# Autodesk Inventor assembly: Horizontal track
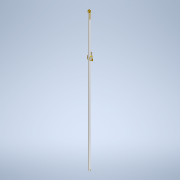
[picture p0: Inventor's stored thumbnail of the model, 180x180]
Saved by Autodesk Inventor 2022 (Build 260153000, 153)
## iProperties
RuleStatus: InUse
Created: 2021-12-23
Part Number: Horizontal track
Document SubType Name: Assembly
Designer: matte
Author: matte
## Documents named in this file (8)
- C:\Users\matte\Documents\GitHub\MDM-Homework\CAD\Horizontal track.iam
- C:\Users\matte\Documents\GitHub\MDM-Homework\CAD\Parts\Ground track\10-081.ipt
- C:\Users\matte\Documents\GitHub\MDM-Homework\CAD\Parts\Ground track\10-240.ipt
- C:\Users\matte\Documents\GitHub\MDM-Homework\CAD\Parts\Ground track\13-106.ipt
- C:\Users\matte\Documents\GitHub\MDM-Homework\CAD\Parts\Ground track\13-505.ipt
- C:\Users\matte\Documents\GitHub\MDM-Homework\CAD\Parts\Ground track\30-404.ipt
- C:\Users\matte\Documents\GitHub\MDM-Homework\CAD\Parts\Ground track\30-407.ipt
- C:\Users\matte\Documents\GitHub\MDM-Homework\CAD\Inventor Component Part Files\08-Linear Application\06-Linear Roller System\04-Components for Bearing Units\02-Bolts\30-006.ipt
## Components (10 placed, 7 different names)
1. 10-081:1 — Allineato:8, Coincidente:7, Allineato:9, Coincidente:8, Allineato:10, Allineato:12
2. 10-240:1 — Allineato:1, Allineato:3, Coincidente:1, Coincidente:2, Coincidente:3, Allineato:4, Allineato:5, Allineato:6, Allineato:12, Allineato:13
3. 13-106:1 — Allineato:1, Allineato:3, Coincidente:1, Coincidente:4, Coincidente:5
4. 13-505:1 — Allineato:5, Coincidente:4, Coincidente:5
5. 30-404:1 — Allineato:8, Coincidente:7, Allineato:9, Allineato:11, Allineato:13
6. 30-407:1 — Coincidente:9, Allineato:14, Allineato:15
7. 13-106:2 — Coincidente:2, Coincidente:3, Allineato:4, Coincidente:6, Allineato:7
8. 13-505:2 — Coincidente:6, Allineato:6, Allineato:7
9. 30-404:2 — Coincidente:8, Allineato:10, Allineato:11, Coincidente:9, Allineato:14, Allineato:15, Inserimento:1
10. 30-006:1 — Inserimento:1
## Relationships (24: Flush 14, Mate 9, Insert 1)
- Allineato:1 [Flush]: 10-240:1 ↔ 13-106:1
- Allineato:3 [Flush]: 10-240:1 ↔ 13-106:1
- Coincidente:1 [Mate]: 10-240:1 ↔ 13-106:1
- Coincidente:2 [Mate]: 10-240:1 ↔ 13-106:2
- Coincidente:3 [Mate]: 10-240:1 ↔ 13-106:2
- Allineato:4 [Flush]: 10-240:1 ↔ 13-106:2
- Allineato:5 [Flush]: 10-240:1 ↔ 13-505:1
- Coincidente:4 [Mate]: 13-106:1 ↔ 13-505:1
- Coincidente:5 [Mate]: 13-106:1 ↔ 13-505:1
- Coincidente:6 [Mate]: 13-106:2 ↔ 13-505:2
- Allineato:6 [Flush]: 10-240:1 ↔ 13-505:2
- Allineato:7 [Flush]: 13-106:2 ↔ 13-505:2
- Allineato:8 [Flush]: 10-081:1 ↔ 30-404:1
- Coincidente:7 [Mate]: 10-081:1 ↔ 30-404:1
- Allineato:9 [Flush] (-40 mm): 10-081:1 ↔ 30-404:1
- Coincidente:8 [Mate]: 10-081:1 ↔ 30-404:2
- Allineato:10 [Flush]: 10-081:1 ↔ 30-404:2
- Allineato:11 [Flush]: 30-404:1 ↔ 30-404:2
- Allineato:12 [Flush] (40 mm): 10-081:1 ↔ 10-240:1
- Allineato:13 [Flush] (-40 mm): 10-240:1 ↔ 30-404:1
- Coincidente:9 [Mate]: 30-407:1 ↔ 30-404:2
- Allineato:14 [Flush]: 30-407:1 ↔ 30-404:2
- Allineato:15 [Flush]: 30-407:1 ↔ 30-404:2
- Inserimento:1: 30-404:2 ↔ 30-006:1
